# Autodesk Inventor assembly: cilindro_0001_001
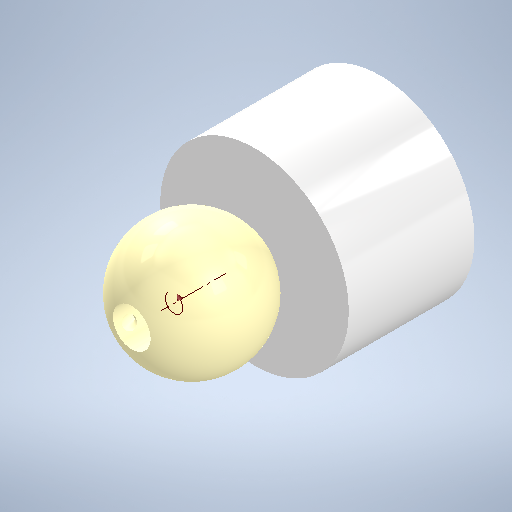
[picture p0: Inventor's stored thumbnail of the model, 512x512]
Saved by Autodesk Inventor 2025.2 (Build 292293000, 293)
## iProperties
Created: 2025-03-26
Part Number: cilindro_0001_001
Document SubType Name: Assembly
Designer: lucas
Author: lucas
## Documents named in this file (3)
- C:\Users\lucas\OneDrive\Documentos\Documentos\Gustavo\Mozangao\Robotica_Fundamentos\Inventor\Seesao5\cilindro_0001_001.iam
- C:\Users\lucas\OneDrive\Documentos\Documentos\Gustavo\Mozangao\Robotica_Fundamentos\Inventor\Seesao5\cilindro_0001_001.ipt
- C:\Users\lucas\OneDrive\Documentos\Documentos\Gustavo\Mozangao\Robotica_Fundamentos\Inventor\Seesao5\Esfera_com_cilindro_0001_001.ipt
## Components (2 placed, 2 different names)
1. cilindro_0001_001:1 — Coincidente:1, Alinhado:1, Coincidente:2, Coincidente:3, Tangente:1
2. Esfera_com_cilindro_0001_001:1 — Coincidente:3, Tangente:1
## Relationships (5: Mate 3, Flush 1, Tangent 1)
- Coincidente:1 [Mate]: cilindro_0001_001:1
- Alinhado:1 [Flush]: cilindro_0001_001:1
- Coincidente:2 [Mate]: cilindro_0001_001:1
- Coincidente:3 [Mate]: cilindro_0001_001:1 ↔ Esfera_com_cilindro_0001_001:1
- Tangente:1: cilindro_0001_001:1 ↔ Esfera_com_cilindro_0001_001:1
